# Autodesk Inventor assembly: Head
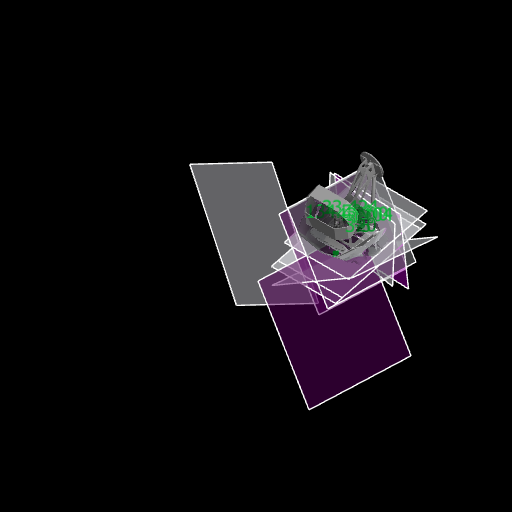
[picture p0: Inventor's stored thumbnail of the model, 512x512]
Saved by Autodesk Inventor 2025.2 (Build 292293000, 293)
## iProperties
Created: 2024-12-17
Part Number: Head
Document SubType Name: Assembly
Designer: valer
Author: valer
## Documents named in this file (41)
- C:\Users\valer\Desktop\str1ker\cad\Head.iam
- C:\Users\valer\Desktop\str1ker\cad\Head.ipt
- C:\Users\valer\Desktop\str1ker\cad\HeadMount.ipt
- C:\Users\valer\Desktop\str1ker\cad\external\HingedThreadedStandoffPart1.ipt
- C:\Users\valer\Desktop\str1ker\cad\external\HingedThreadedStandoffPart2.ipt
- C:\Users\valer\Desktop\str1ker\cad\ShaftD6FemaleCollar.ipt
- C:\Users\valer\Desktop\str1ker\cad\external\ShaftD6-2101-0006-0160.ipt
- C:\Users\valer\Desktop\str1ker\cad\TongueMount.ipt
- C:\Users\valer\Desktop\str1ker\cad\external\SetScrewLiteHub-1308-0016-0006.ipt
- C:\Users\valer\Desktop\str1ker\cad\external\ShaftD6-Short-2101-0006-0020.ipt
- C:\Users\valer\Desktop\str1ker\cad\external\UJoint6D\UJoint6D-Body-4003-1006-1006.ipt
- C:\Users\valer\Desktop\str1ker\cad\external\UJoint6D\UJoint6D-Screw.ipt
- C:\Users\valer\Desktop\str1ker\cad\external\ShaftD6-2100-0006-0200.ipt
- C:\Users\valer\Desktop\str1ker\cad\external\ShaftD6-2101-0006-0140.ipt
- C:\Users\valer\Desktop\str1ker\cad\external\LinearBearing-1612-0612-0035.ipt
- C:\Users\valer\Desktop\str1ker\cad\external\ClampingHub1301-0016-0012.ipt
- C:\Users\valer\Desktop\str1ker\cad\external\ShaftClamp6-6058N14.ipt
- C:\Users\valer\Desktop\str1ker\cad\external\TongueSpeaker.ipt
- C:\Users\valer\Desktop\str1ker\cad\TongueSideLid.ipt
- C:\Users\valer\Desktop\str1ker\cad\TongueSideLidMirror.ipt
- C:\Users\valer\Desktop\str1ker\cad\NoseMount.ipt
- C:\Users\valer\Desktop\str1ker\cad\JawMount.ipt
- C:\Users\valer\Desktop\str1ker\cad\Visor.ipt
- C:\Users\valer\Desktop\str1ker\cad\NeckBase.ipt
- C:\Users\valer\Desktop\str1ker\cad\external\HeadServo\M3RCServoMountBracket.ipt
- C:\Users\valer\Desktop\str1ker\cad\external\NeckActuator\1610-50H-2KG-12V-B07-Body.ipt
- C:\Users\valer\Desktop\str1ker\cad\external\NeckActuator\1610-50H-2KG-12V-B07-Shaft.ipt
- C:\Users\valer\Desktop\str1ker\cad\external\59935K12_Ball Joint Rod End.ipt
- C:\Users\valer\Desktop\str1ker\cad\external\NexusRobot14mmKeywayHub.ipt
- C:\Users\valer\Desktop\str1ker\cad\external\HeadServo\PerfectPass56KG.ipt
- C:\Users\valer\Desktop\str1ker\cad\NeckCover.ipt
- C:\Users\valer\Desktop\str1ker\cad\NeckBracket.ipt
- C:\Users\valer\Desktop\str1ker\cad\NeckBracketMirror.ipt
- C:\Users\valer\Desktop\str1ker\cad\external\4005-0016-0001 Half.iam
- C:\Users\valer\Desktop\str1ker\cad\external\1505-0032-0160.ipt
- C:\Users\valer\Desktop\str1ker\cad\external\4005-0016-0001 Ball.ipt
- C:\Users\valer\Desktop\str1ker\cad\external\1221-0032-0002.ipt
- C:\Users\valer\Desktop\str1ker\cad\external\UJoint6D\UJoint6D-CenterDrive-4003-1006-1006.ipt
- C:\Users\valer\Desktop\str1ker\cad\DepthSensor.iam
- C:\Users\valer\Desktop\str1ker\cad\external\1204-0001-0001.ipt
- C:\Users\valer\Desktop\str1ker\cad\CameraMount.ipt
## Components (85 placed, 40 different names)
1. Head:1 — Flush:1, Flush:2, Mate:1, Flush:3, Mate:4, Mate:5, Mate:6, Mate:7, Mate:8, Mate:9, Mate:10, Mate:11, Mate:12, Mate:13, Mate:14, Mate:15, Mate:16, Mate:17, Mate:18, Mate:19, Mate:20, Mate:59, Angle:13, Mate:89, Mate:90, Flush:13, Mate:119, Mate:121, Flush:15, Flush:16, Flush:17, Flush:18, Flush:19, Mate:124, Mate:125, Mate:126, Mate:127, Mate:128, Mate:129, Flush:20, Mate:131, Mate:132, Mate:133, Flush:157
2. HeadMount:1 — Flush:4, Flush:5, Angle:18, Mate:89, Mate:90, Angle:20, Angle:22, Angle:26, Angle:28, Angle:32, Mate:105, Mate:107, Mate:109, Mate:111, Mate:113, Mate:115, Flush:158, Mate:178, Angle:37, Mate:344, Mate:347, Mate:376, Mate:377, Mate:384, Mate:387, Angle:57, Mate:447, Mate:448, Mate:449, Mate:452, Mate:458, Mate:465, Mate:466, Angle:60, Mate:473, Angle:62, Angle:63, Mate:492, Mate:493, Mate:494
3. HingedThreadedStandoffPart1:1 — Mate:4, Mate:5, Mate:25, Mate:26
4. HingedThreadedStandoffPart1:2 — Mate:6, Mate:7, Mate:36, Mate:39
5. HingedThreadedStandoffPart1:3 — Mate:8, Mate:9, Mate:37, Mate:38
6. HingedThreadedStandoffPart1:4 — Mate:10, Mate:11, Mate:23, Mate:24
7. HingedThreadedStandoffPart1:5 — Mate:12, Mate:13, Mate:27, Mate:28
8. HingedThreadedStandoffPart1:6 — Mate:16, Mate:17, Mate:29, Mate:40
9. HingedThreadedStandoffPart1:7 — Mate:14, Mate:15, Mate:30, Mate:31
10. HingedThreadedStandoffPart1:8 — Mate:18, Mate:19, Mate:32, Mate:34
11. HingedThreadedStandoffPart1:9 — Mate:20, Mate:33, Mate:35, Mate:59
12. HingedThreadedStandoffPart2:4 — Mate:23, Mate:24, Flush:7, Flush:8
13. HingedThreadedStandoffPart2:5 — Mate:25, Mate:26, Flush:8, Mate:68
14. HingedThreadedStandoffPart2:6 — Mate:27, Mate:28, Flush:7, Flush:10, Mate:69
15. HingedThreadedStandoffPart2:7 — Mate:29, Mate:40, Mate:45, Mate:47
16. HingedThreadedStandoffPart2:8 — Mate:30, Mate:31, Mate:46, Mate:48
17. HingedThreadedStandoffPart2:9 — Mate:32, Mate:34, Mate:49, Mate:52
18. HingedThreadedStandoffPart2:10 — Mate:33, Mate:35, Mate:50, Mate:51
19. HingedThreadedStandoffPart2:11 — Mate:36, Mate:39, Mate:41, Mate:42
20. HingedThreadedStandoffPart2:12 — Mate:37, Mate:38, Mate:43, Mate:44
21. ShaftD6-2100-0006-0200:1 — Mate:87, Angle:17, Mate:88, Angle:18, Mate:108
22. ShaftD6FemaleCollar:1 — Mate:41, Mate:42, Mate:87, Angle:17, Mate:88
23. ShaftD6FemaleCollar:2 — Mate:43, Mate:44, Mate:91, Mate:92
24. ShaftD6FemaleCollar:3 — Mate:45, Mate:47, Mate:95, Mate:96, Angle:23
25. ShaftD6FemaleCollar:4 — Mate:46, Mate:48, Mate:93, Mate:94, Angle:21
26. ShaftD6FemaleCollar:5 — Mate:49, Mate:52, Mate:99, Mate:100, Angle:30
27. ShaftD6FemaleCollar:6 — Mate:50, Mate:51, Mate:97, Mate:98, Angle:27
28. TongueMount:1 — Mate:66, Mate:67, Angle:11, Mate:68, Mate:69, Mate:71
29. SetScrewLiteHub-1308-0016-0006:1 — Mate:66, Mate:67, Angle:11, Mate:70, Mate:73, Angle:61
30. ShaftD6-Short-2101-0006-0020:1 — Mate:70, Mate:71, Mate:72, Angle:12
31. UJoint6D-Body-4003-1006-1006:1 — Mate:72, Mate:73, Angle:12, Mate:76, Mate:77, Mate:78, Mate:79, Angle:61
32. UJoint6D-Screw:1 — Mate:82, Mate:83
33. UJoint6D-Screw:2 — Mate:76, Mate:77
34. UJoint6D-Screw:3 — Mate:78, Mate:79, Mate:474
35. UJoint6D-Body-4003-1006-1006:2 — Angle:13, Mate:82, Mate:83, Mate:84, Mate:85, Mate:86, Angle:14, Flush:12
36. UJoint6D-Screw:4 — Mate:84, Mate:85, Mate:476
37. ShaftD6-2101-0006-0160:7 — Mate:86, Angle:14, Flush:12, Mate:101, Mate:473, Mate:477, Flush:187
38. ShaftD6-2100-0006-0200:2 — Mate:91, Mate:92, Angle:19, Angle:20, Mate:110
39. ShaftD6-2101-0006-0140:1 — Mate:93, Mate:94, Angle:21, Angle:22, Angle:24, Mate:104
40. ShaftD6-2101-0006-0140:2 — Mate:95, Mate:96, Angle:23, Angle:25, Angle:26, Mate:106
41. ShaftD6-2101-0006-0140:3 — Mate:97, Mate:98, Angle:27, Angle:28, Angle:29, Mate:112
42. ShaftD6-2101-0006-0140:4 — Mate:99, Mate:100, Angle:30, Angle:31, Angle:32, Mate:114
43. LinearBearing-1612-0612-0035:1 — Mate:101, Mate:103, Flush:160
44. ClampingHub1301-0016-0012:1 — Mate:103, Flush:160, Angle:37, Mate:347
45. ShaftClamp6-6058N14:1 — Mate:106, Mate:107
46. ShaftClamp6-6058N14:2 — Mate:104, Mate:105
47. ShaftClamp6-6058N14:3 — Mate:108, Mate:109
48. ShaftClamp6-6058N14:4 — Mate:110, Mate:111
49. ShaftClamp6-6058N14:5 — Mate:114, Mate:115
50. ShaftClamp6-6058N14:6 — Mate:112, Mate:113
51. TongueSpeaker:1 — Mate:119, Mate:122, Mate:123
52. TongueSpeaker:2 — Mate:121, Mate:130
53. TongueSideLid:1 — Mate:124, Mate:125, Mate:126
54. TongueSideLidMirror:1 — Mate:127, Mate:128, Mate:129, Mate:130
55. NoseMount:1 — Flush:21, Mate:131, Mate:132, Mate:133
56. JawMount:1 — Flush:22
57. Visor:1 — Flush:157, Flush:158, Mate:178
58. M3RCServoMountBracket:1 — Mate:344, Mate:449, Mate:450, Mate:451, Mate:452, Angle:59, Mate:453
59. 1610-50H-2KG-12V-B07-Body:1 — Cylindrical:1, Mate:378, Mate:379, Mate:482
60. 1610-50H-2KG-12V-B07-Shaft:1 — Cylindrical:1, Mate:380, Mate:382, Mate:482
61. 1610-50H-2KG-12V-B07-Body:2 — Mate:385, Mate:386, Mate:390
62. 59935K12_Ball Joint Rod End:1 — Mate:378, Mate:379, Mate:471
63. 59935K12_Ball Joint Rod End:2 — Mate:385, Mate:386, Mate:470
64. 59935K12_Ball Joint Rod End:3 — Mate:376, Mate:380, Mate:382, Mate:384
65. 59935K12_Ball Joint Rod End:4 — Mate:377, Mate:387, Mate:388, Mate:389
66. 1610-50H-2KG-12V-B07-Shaft:2 — Mate:388, Mate:389, Mate:390
67. NexusRobot14mmKeywayHub:1 — Mate:407, Mate:472, Angle:60
68. NeckBase:1 — Mate:407, Angle:57, Mate:434, Mate:458, Mate:472, Mate:483
69. NeckCover:1 — Mate:463, Mate:466
70. NeckBracket:1 — Mate:434, Flush:185, Flush:186, Mate:461, Mate:471, Mate:478, Mate:483
71. NeckBracketMirror:1 — Flush:185, Flush:186, Mate:462, Mate:463, Mate:464, Mate:470, Mate:479
72. 4005-0016-0001 Half:1 [sub-assembly] — Mate:438, Mate:448, Mate:453, Mate:454, Mate:455, Mate:480
73. 1505-0032-0160:1 — Mate:438, Mate:447, Mate:480
74. 4005-0016-0001 Half:2 [sub-assembly] — Mate:456, Mate:457, Mate:481
75. 1505-0032-0160:2 — Mate:459, Mate:460, Mate:481
76. PerfectPass56KG:1 — Mate:450, Mate:451, Angle:59
77. 4005-0016-0001 Ball:1 — Mate:454, Mate:455, Mate:456, Mate:457
78. 1221-0032-0002:1 — Mate:459, Mate:460, Mate:461, Mate:462, Mate:478, Mate:479
79. NeckCover:2 — Mate:464, Mate:465
80. UJoint6D-CenterDrive-4003-1006-1006:1 — Mate:474, Mate:476
81. ShaftClamp6-6058N14:7 — Mate:477, Flush:187
82. DepthSensor:1 [sub-assembly] — Mate:490, Mate:491, Mate:495, Mate:497
83. 1204-0001-0001:1 — Angle:62, Mate:490, Mate:497, Mate:498
84. 1204-0001-0001:2 — Angle:63, Mate:495, Mate:496
85. CameraMount:1 — Mate:492, Mate:493, Mate:494, Mate:496, Mate:498
## Relationships (224: Mate 170, Angle 27, Flush 24, Symmetry 2, CylindricalJoint 1)
- Flush:1: Head:1
- Flush:2: Head:1
- Mate:1: Head:1
- Flush:3: Head:1
- Flush:4: HeadMount:1
- Flush:5: HeadMount:1
- Mate:4: Head:1 ↔ HingedThreadedStandoffPart1:1
- Mate:5: Head:1 ↔ HingedThreadedStandoffPart1:1
- Mate:6: Head:1 ↔ HingedThreadedStandoffPart1:2
- Mate:7: Head:1 ↔ HingedThreadedStandoffPart1:2
- Mate:8: Head:1 ↔ HingedThreadedStandoffPart1:3
- Mate:9: Head:1 ↔ HingedThreadedStandoffPart1:3
- Mate:10: Head:1 ↔ HingedThreadedStandoffPart1:4
- Mate:11: Head:1 ↔ HingedThreadedStandoffPart1:4
- Mate:12: Head:1 ↔ HingedThreadedStandoffPart1:5
- Mate:13: Head:1 ↔ HingedThreadedStandoffPart1:5
- Mate:14: Head:1 ↔ HingedThreadedStandoffPart1:7
- Mate:15: Head:1 ↔ HingedThreadedStandoffPart1:7
- Mate:16: Head:1 ↔ HingedThreadedStandoffPart1:6
- Mate:17: Head:1 ↔ HingedThreadedStandoffPart1:6
- Mate:18: Head:1 ↔ HingedThreadedStandoffPart1:8
- Mate:19: Head:1 ↔ HingedThreadedStandoffPart1:8
- Mate:20: Head:1 ↔ HingedThreadedStandoffPart1:9
- Mate:23: HingedThreadedStandoffPart1:4 ↔ HingedThreadedStandoffPart2:4
- Mate:24: HingedThreadedStandoffPart1:4 ↔ HingedThreadedStandoffPart2:4
- Mate:25: HingedThreadedStandoffPart1:1 ↔ HingedThreadedStandoffPart2:5
- Mate:26: HingedThreadedStandoffPart1:1 ↔ HingedThreadedStandoffPart2:5
- Mate:27: HingedThreadedStandoffPart1:5 ↔ HingedThreadedStandoffPart2:6
- Mate:28: HingedThreadedStandoffPart1:5 ↔ HingedThreadedStandoffPart2:6
- Mate:29: HingedThreadedStandoffPart1:6 ↔ HingedThreadedStandoffPart2:7
- Mate:30: HingedThreadedStandoffPart1:7 ↔ HingedThreadedStandoffPart2:8
- Mate:31: HingedThreadedStandoffPart1:7 ↔ HingedThreadedStandoffPart2:8
- Mate:32: HingedThreadedStandoffPart1:8 ↔ HingedThreadedStandoffPart2:9
- Mate:33: HingedThreadedStandoffPart1:9 ↔ HingedThreadedStandoffPart2:10
- Mate:34: HingedThreadedStandoffPart1:8 ↔ HingedThreadedStandoffPart2:9
- Mate:35: HingedThreadedStandoffPart1:9 ↔ HingedThreadedStandoffPart2:10
- Mate:36: HingedThreadedStandoffPart1:2 ↔ HingedThreadedStandoffPart2:11
- Mate:37: HingedThreadedStandoffPart1:3 ↔ HingedThreadedStandoffPart2:12
- Mate:38: HingedThreadedStandoffPart1:3 ↔ HingedThreadedStandoffPart2:12
- Mate:39: HingedThreadedStandoffPart1:2 ↔ HingedThreadedStandoffPart2:11
- Mate:40: HingedThreadedStandoffPart1:6 ↔ HingedThreadedStandoffPart2:7
- Flush:7: HingedThreadedStandoffPart2:4 ↔ HingedThreadedStandoffPart2:6
- Flush:8: HingedThreadedStandoffPart2:4 ↔ HingedThreadedStandoffPart2:5
- Mate:41: HingedThreadedStandoffPart2:11 ↔ ShaftD6FemaleCollar:1
- Mate:42: HingedThreadedStandoffPart2:11 ↔ ShaftD6FemaleCollar:1
- Mate:43: HingedThreadedStandoffPart2:12 ↔ ShaftD6FemaleCollar:2
- Mate:44: HingedThreadedStandoffPart2:12 ↔ ShaftD6FemaleCollar:2
- Mate:45: HingedThreadedStandoffPart2:7 ↔ ShaftD6FemaleCollar:3
- Mate:46: HingedThreadedStandoffPart2:8 ↔ ShaftD6FemaleCollar:4
- Mate:47: HingedThreadedStandoffPart2:7 ↔ ShaftD6FemaleCollar:3
- Mate:48: HingedThreadedStandoffPart2:8 ↔ ShaftD6FemaleCollar:4
- Mate:49: HingedThreadedStandoffPart2:9 ↔ ShaftD6FemaleCollar:5
- Mate:50: HingedThreadedStandoffPart2:10 ↔ ShaftD6FemaleCollar:6
- Mate:51: HingedThreadedStandoffPart2:10 ↔ ShaftD6FemaleCollar:6
- Mate:52: HingedThreadedStandoffPart2:9 ↔ ShaftD6FemaleCollar:5
- Mate:59: Head:1 ↔ HingedThreadedStandoffPart1:9
- Flush:10: HingedThreadedStandoffPart2:6
- Mate:66: TongueMount:1 ↔ SetScrewLiteHub-1308-0016-0006:1
- Mate:67: TongueMount:1 ↔ SetScrewLiteHub-1308-0016-0006:1
- Angle:11 (0 deg): TongueMount:1 ↔ SetScrewLiteHub-1308-0016-0006:1
- Mate:68: HingedThreadedStandoffPart2:5 ↔ TongueMount:1
- Mate:69: HingedThreadedStandoffPart2:6 ↔ TongueMount:1
- Mate:70: SetScrewLiteHub-1308-0016-0006:1 ↔ ShaftD6-Short-2101-0006-0020:1
- Mate:71: TongueMount:1 ↔ ShaftD6-Short-2101-0006-0020:1
- Mate:72: ShaftD6-Short-2101-0006-0020:1 ↔ UJoint6D-Body-4003-1006-1006:1
- Mate:73: SetScrewLiteHub-1308-0016-0006:1 ↔ UJoint6D-Body-4003-1006-1006:1
- Angle:12 (0 deg): ShaftD6-Short-2101-0006-0020:1 ↔ UJoint6D-Body-4003-1006-1006:1
- Mate:76: UJoint6D-Body-4003-1006-1006:1 ↔ UJoint6D-Screw:2
- Mate:77: UJoint6D-Body-4003-1006-1006:1 ↔ UJoint6D-Screw:2
- Mate:78: UJoint6D-Body-4003-1006-1006:1 ↔ UJoint6D-Screw:3
- Mate:79: UJoint6D-Body-4003-1006-1006:1 ↔ UJoint6D-Screw:3
- Angle:13 (0 deg): Head:1 ↔ UJoint6D-Body-4003-1006-1006:2
- Mate:82: UJoint6D-Screw:1 ↔ UJoint6D-Body-4003-1006-1006:2
- Mate:83: UJoint6D-Screw:1 ↔ UJoint6D-Body-4003-1006-1006:2
- Mate:84: UJoint6D-Body-4003-1006-1006:2 ↔ UJoint6D-Screw:4
- Mate:85: UJoint6D-Body-4003-1006-1006:2 ↔ UJoint6D-Screw:4
- Mate:86: UJoint6D-Body-4003-1006-1006:2 ↔ ShaftD6-2101-0006-0160:7
- Angle:14 (180 deg): UJoint6D-Body-4003-1006-1006:2 ↔ ShaftD6-2101-0006-0160:7
- Flush:12: UJoint6D-Body-4003-1006-1006:2 ↔ ShaftD6-2101-0006-0160:7
- Mate:87: ShaftD6-2100-0006-0200:1 ↔ ShaftD6FemaleCollar:1
- Angle:17 (0 deg): ShaftD6-2100-0006-0200:1 ↔ ShaftD6FemaleCollar:1
- Mate:88: ShaftD6-2100-0006-0200:1 ↔ ShaftD6FemaleCollar:1
- Angle:18 (0 deg): HeadMount:1 ↔ ShaftD6-2100-0006-0200:1
- Mate:89: Head:1 ↔ HeadMount:1
- Mate:90: Head:1 ↔ HeadMount:1
- Mate:91: ShaftD6FemaleCollar:2 ↔ ShaftD6-2100-0006-0200:2
- Mate:92: ShaftD6FemaleCollar:2 ↔ ShaftD6-2100-0006-0200:2
- Angle:19 (0 deg): ShaftD6-2100-0006-0200:2
- Angle:20 (0 deg): HeadMount:1 ↔ ShaftD6-2100-0006-0200:2
- Mate:93: ShaftD6FemaleCollar:4 ↔ ShaftD6-2101-0006-0140:1
- Mate:94: ShaftD6FemaleCollar:4 ↔ ShaftD6-2101-0006-0140:1
- Angle:21 (0 deg): ShaftD6FemaleCollar:4 ↔ ShaftD6-2101-0006-0140:1
- Angle:22 (0 deg): HeadMount:1 ↔ ShaftD6-2101-0006-0140:1
- Mate:95: ShaftD6FemaleCollar:3 ↔ ShaftD6-2101-0006-0140:2
- Mate:96: ShaftD6FemaleCollar:3 ↔ ShaftD6-2101-0006-0140:2
- Angle:23 (0 deg): ShaftD6FemaleCollar:3 ↔ ShaftD6-2101-0006-0140:2
- Angle:24 (180 deg): ShaftD6-2101-0006-0140:1
- Angle:25 (180 deg): ShaftD6-2101-0006-0140:2
- Angle:26 (0 deg): HeadMount:1 ↔ ShaftD6-2101-0006-0140:2
- Mate:97: ShaftD6FemaleCollar:6 ↔ ShaftD6-2101-0006-0140:3
- Mate:98: ShaftD6FemaleCollar:6 ↔ ShaftD6-2101-0006-0140:3
- Angle:27 (0 deg): ShaftD6FemaleCollar:6 ↔ ShaftD6-2101-0006-0140:3
- Angle:28 (0 deg): HeadMount:1 ↔ ShaftD6-2101-0006-0140:3
- Angle:29 (0 deg): ShaftD6-2101-0006-0140:3
- Mate:99: ShaftD6FemaleCollar:5 ↔ ShaftD6-2101-0006-0140:4
- Mate:100: ShaftD6FemaleCollar:5 ↔ ShaftD6-2101-0006-0140:4
- Angle:30 (0 deg): ShaftD6FemaleCollar:5 ↔ ShaftD6-2101-0006-0140:4
- Angle:31 (0 deg): ShaftD6-2101-0006-0140:4
- Angle:32 (0 deg): HeadMount:1 ↔ ShaftD6-2101-0006-0140:4
- Mate:101: ShaftD6-2101-0006-0160:7 ↔ LinearBearing-1612-0612-0035:1
- Mate:103: LinearBearing-1612-0612-0035:1 ↔ ClampingHub1301-0016-0012:1
- Mate:104: ShaftD6-2101-0006-0140:1 ↔ ShaftClamp6-6058N14:2
- Mate:105: HeadMount:1 ↔ ShaftClamp6-6058N14:2
- Mate:106: ShaftD6-2101-0006-0140:2 ↔ ShaftClamp6-6058N14:1
- Mate:107: HeadMount:1 ↔ ShaftClamp6-6058N14:1
- Mate:108: ShaftD6-2100-0006-0200:1 ↔ ShaftClamp6-6058N14:3
- Mate:109: HeadMount:1 ↔ ShaftClamp6-6058N14:3
- Mate:110: ShaftD6-2100-0006-0200:2 ↔ ShaftClamp6-6058N14:4
- Mate:111: HeadMount:1 ↔ ShaftClamp6-6058N14:4
- Mate:112: ShaftD6-2101-0006-0140:3 ↔ ShaftClamp6-6058N14:6
- Mate:113: HeadMount:1 ↔ ShaftClamp6-6058N14:6
- Mate:114: ShaftD6-2101-0006-0140:4 ↔ ShaftClamp6-6058N14:5
- Mate:115: HeadMount:1 ↔ ShaftClamp6-6058N14:5
- Flush:13: Head:1
- Mate:119: Head:1 ↔ TongueSpeaker:1
- Mate:121: Head:1 ↔ TongueSpeaker:2
- Flush:15: Head:1
- Flush:16: Head:1
- Symmetry:1
- Mate:122: TongueSpeaker:1
- Flush:17: Head:1
- Flush:18: Head:1
- Symmetry:2
- Mate:123: TongueSpeaker:1
- Flush:19: Head:1
- Mate:124: Head:1 ↔ TongueSideLid:1
- Mate:125: Head:1 ↔ TongueSideLid:1
- Mate:126: Head:1 ↔ TongueSideLid:1
- Mate:127: Head:1 ↔ TongueSideLidMirror:1
- Mate:128: Head:1 ↔ TongueSideLidMirror:1
- Mate:129: Head:1 ↔ TongueSideLidMirror:1
- Mate:130: TongueSpeaker:2 ↔ TongueSideLidMirror:1
- Flush:20: Head:1
- Flush:21: NoseMount:1
- Mate:131: Head:1 ↔ NoseMount:1
- Mate:132: Head:1 ↔ NoseMount:1
- Mate:133: Head:1 ↔ NoseMount:1
- Flush:22: JawMount:1
- Flush:157: Head:1 ↔ Visor:1
- Flush:158: HeadMount:1 ↔ Visor:1
- Mate:178: HeadMount:1 ↔ Visor:1
- Flush:160: LinearBearing-1612-0612-0035:1 ↔ ClampingHub1301-0016-0012:1
- Angle:37 (0 deg): HeadMount:1 ↔ ClampingHub1301-0016-0012:1
- Mate:344: HeadMount:1 ↔ M3RCServoMountBracket:1
- Mate:347: HeadMount:1 ↔ ClampingHub1301-0016-0012:1
- Mate:376: HeadMount:1 ↔ 59935K12_Ball Joint Rod End:3
- Mate:377: HeadMount:1 ↔ 59935K12_Ball Joint Rod End:4
- Cylindrical:1: 1610-50H-2KG-12V-B07-Body:1 ↔ 1610-50H-2KG-12V-B07-Shaft:1
- Mate:378: 1610-50H-2KG-12V-B07-Body:1 ↔ 59935K12_Ball Joint Rod End:1
- Mate:379: 1610-50H-2KG-12V-B07-Body:1 ↔ 59935K12_Ball Joint Rod End:1
- Mate:380: 1610-50H-2KG-12V-B07-Shaft:1 ↔ 59935K12_Ball Joint Rod End:3
- Mate:382: 1610-50H-2KG-12V-B07-Shaft:1 ↔ 59935K12_Ball Joint Rod End:3
- Mate:384 (8 mm): HeadMount:1 ↔ 59935K12_Ball Joint Rod End:3
- Mate:385: 1610-50H-2KG-12V-B07-Body:2 ↔ 59935K12_Ball Joint Rod End:2
- Mate:386: 1610-50H-2KG-12V-B07-Body:2 ↔ 59935K12_Ball Joint Rod End:2
- Mate:387 (8 mm): HeadMount:1 ↔ 59935K12_Ball Joint Rod End:4
- Mate:388: 59935K12_Ball Joint Rod End:4 ↔ 1610-50H-2KG-12V-B07-Shaft:2
- Mate:389: 59935K12_Ball Joint Rod End:4 ↔ 1610-50H-2KG-12V-B07-Shaft:2
- Mate:390: 1610-50H-2KG-12V-B07-Body:2 ↔ 1610-50H-2KG-12V-B07-Shaft:2
- Mate:407: NexusRobot14mmKeywayHub:1 ↔ NeckBase:1
- Angle:57 (0 deg): HeadMount:1 ↔ NeckBase:1
- Mate:434: NeckBase:1 ↔ NeckBracket:1
- Flush:185: NeckBracket:1 ↔ NeckBracketMirror:1
- Flush:186: NeckBracket:1 ↔ NeckBracketMirror:1
- Mate:438: 4005-0016-0001 Half:1 ↔ 1505-0032-0160:1
- [Mate]: 4005-0016-0001 Half:2 ↔ 1505-0032-0160:2
- Mate:447: HeadMount:1 ↔ 1505-0032-0160:1
- Mate:448: HeadMount:1 ↔ 4005-0016-0001 Half:1
- Mate:449: HeadMount:1 ↔ M3RCServoMountBracket:1
- Mate:450: M3RCServoMountBracket:1 ↔ PerfectPass56KG:1
- Mate:451: M3RCServoMountBracket:1 ↔ PerfectPass56KG:1
- Mate:452: HeadMount:1 ↔ M3RCServoMountBracket:1
- Angle:59 (0 deg): M3RCServoMountBracket:1 ↔ PerfectPass56KG:1
- Mate:453 (13 mm): M3RCServoMountBracket:1 ↔ 4005-0016-0001 Half:1
- Mate:454: 4005-0016-0001 Half:1 ↔ 4005-0016-0001 Ball:1
- Mate:455 (0.25 mm): 4005-0016-0001 Half:1 ↔ 4005-0016-0001 Ball:1
- Mate:456: 4005-0016-0001 Half:2 ↔ 4005-0016-0001 Ball:1
- Mate:457 (0.25 mm): 4005-0016-0001 Half:2 ↔ 4005-0016-0001 Ball:1
- Mate:458: HeadMount:1 ↔ NeckBase:1
- Mate:459: 1505-0032-0160:2 ↔ 1221-0032-0002:1
- Mate:460: 1505-0032-0160:2 ↔ 1221-0032-0002:1
- Mate:461: NeckBracket:1 ↔ 1221-0032-0002:1
- Mate:462: NeckBracketMirror:1 ↔ 1221-0032-0002:1
- Mate:463: NeckCover:1 ↔ NeckBracketMirror:1
- Mate:464: NeckBracketMirror:1 ↔ NeckCover:2
- Mate:465: HeadMount:1 ↔ NeckCover:2
- Mate:466: HeadMount:1 ↔ NeckCover:1
- Mate:470: 59935K12_Ball Joint Rod End:2 ↔ NeckBracketMirror:1
- Mate:471: 59935K12_Ball Joint Rod End:1 ↔ NeckBracket:1
- Mate:472: NexusRobot14mmKeywayHub:1 ↔ NeckBase:1
- Angle:60 (0 deg): HeadMount:1 ↔ NexusRobot14mmKeywayHub:1
- Mate:473: HeadMount:1 ↔ ShaftD6-2101-0006-0160:7
- Mate:474: UJoint6D-Screw:3 ↔ UJoint6D-CenterDrive-4003-1006-1006:1
- Mate:476: UJoint6D-Screw:4 ↔ UJoint6D-CenterDrive-4003-1006-1006:1
- Mate:477: ShaftD6-2101-0006-0160:7 ↔ ShaftClamp6-6058N14:7
- Flush:187 (2 mm): ShaftD6-2101-0006-0160:7 ↔ ShaftClamp6-6058N14:7
- Angle:61 (0 deg): SetScrewLiteHub-1308-0016-0006:1 ↔ UJoint6D-Body-4003-1006-1006:1
- Mate:478: NeckBracket:1 ↔ 1221-0032-0002:1
- Mate:479: NeckBracketMirror:1 ↔ 1221-0032-0002:1
- Mate:480: 4005-0016-0001 Half:1 ↔ 1505-0032-0160:1
- Mate:481: 4005-0016-0001 Half:2 ↔ 1505-0032-0160:2
- Mate:482: 1610-50H-2KG-12V-B07-Body:1 ↔ 1610-50H-2KG-12V-B07-Shaft:1
- Mate:483: NeckBase:1 ↔ NeckBracket:1
- Angle:62 (0 deg): HeadMount:1 ↔ 1204-0001-0001:1
- Angle:63 (0 deg): HeadMount:1 ↔ 1204-0001-0001:2
- Mate:490: DepthSensor:1 ↔ 1204-0001-0001:1
- Mate:491: DepthSensor:1
- Mate:492: HeadMount:1 ↔ CameraMount:1
- Mate:493: HeadMount:1 ↔ CameraMount:1
- Mate:494: HeadMount:1 ↔ CameraMount:1
- Mate:495: DepthSensor:1 ↔ 1204-0001-0001:2
- Mate:496: 1204-0001-0001:2 ↔ CameraMount:1
- Mate:497: DepthSensor:1 ↔ 1204-0001-0001:1
- Mate:498: 1204-0001-0001:1 ↔ CameraMount:1
## Named parameters: d832_d824 = 0 mm
